# Autodesk Inventor assembly: Bio Assembly Skiba
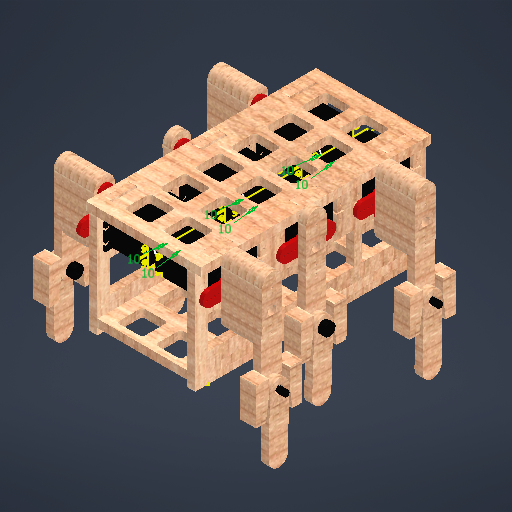
[picture p0: Inventor's stored thumbnail of the model, 512x512]
Saved by Autodesk Inventor 2026.2 (Build 302298000, 298)
## iProperties
Created: 2025-11-09
Part Number: Bio Assembly Skiba
Document SubType Name: Assembly
Designer: Nick
Author: Nick
## Documents named in this file (11)
- C:\Users\Nick\Downloads\CAD\Inventor\MMAE 232 Homeworks\Bio\Bio Assembly Skiba.iam
- C:\Users\Nick\Downloads\CAD\Inventor\MMAE 232 Homeworks\Bio\CAD Parts\Base-Skiba.ipt
- C:\Users\Nick\Downloads\CAD\Inventor\MMAE 232 Homeworks\Bio\CAD Parts\Servo Wall Skiba.ipt
- C:\Users\Nick\Downloads\CAD\Inventor\MMAE 232 Homeworks\Bio\CAD Parts\Bio Servo Skiba.ipt
- C:\Users\Nick\Downloads\CAD\Inventor\MMAE 232 Homeworks\Bio\CAD Parts\Servo Horn Skiba.ipt
- C:\Users\Nick\Downloads\CAD\Inventor\MMAE 232 Homeworks\Bio\CAD Parts\Roof Skiba.ipt
- C:\Users\Nick\Downloads\CAD\Inventor\MMAE 232 Homeworks\Bio\CAD Parts\Spacer Skiba.ipt
- C:\Users\Nick\Downloads\CAD\Inventor\MMAE 232 Homeworks\Bio\CAD Parts\Upper Leg Skiba.ipt
- C:\Users\Nick\Downloads\CAD\Inventor\MMAE 232 Homeworks\Bio\CAD Parts\Stop Skiba.ipt
- C:\Users\Nick\Downloads\CAD\Inventor\MMAE 232 Homeworks\Bio\CAD Parts\Lower Leg Skiba.ipt
- C:\Users\Nick\Downloads\CAD\Inventor\MMAE 232 Homeworks\Bio\CAD Parts\93897A255_Nylon Shoulder Screws (Short Screw) Skiba.ipt
## Components (62 placed, 10 different names)
1. Base-Skiba:1 — Flush:14, Mate:65, Flush:23, Flush:24, Flush:25, Flush:26, Mate:66
2. Servo Wall Skiba:1 — Mate:3, Mate:4, Mate:5, Mate:65, Flush:23, Flush:24, Flush:27, Mate:67, Flush:28
3. Servo Horn Skiba:2 — Mate:16, Mate:17, Mate:84, Mate:85, Mate:86
4. Servo Wall Skiba:2 — Flush:14, Mate:36, Mate:37, Mate:38, Flush:25, Flush:26, Mate:66
5. Servo Horn Skiba:5 — Mate:41, Mate:42, Mate:108, Mate:109, Mate:110
6. Roof Skiba:1 — Flush:27, Mate:67, Flush:28
7. Upper Leg Skiba:2 — Mate:84, Mate:85, Mate:86, Mate:87, Flush:35, Flush:36, Mate:88, Mate:89, Mate:117, Flush:47, Flush:48
8. Stop Skiba:2 — Mate:87, Flush:35, Flush:36
9. 93897A255_Nylon Shoulder Screws (Short Screw) Skiba:2 — Mate:90, Mate:91
10. Lower Leg Skiba:2 — Mate:88, Mate:89, Mate:90, Mate:91
11. Upper Leg Skiba:5 — Mate:108, Mate:109, Mate:110, Mate:111, Flush:43, Flush:44, Mate:112, Mate:113, Mate:120, Flush:53, Flush:54
12. Stop Skiba:5 — Mate:111, Flush:43, Flush:44
13. Lower Leg Skiba:5 — Mate:112, Mate:113, Mate:114, Mate:115
14. 93897A255_Nylon Shoulder Screws (Short Screw) Skiba:5 — Mate:114, Mate:115
15. Stop Skiba:7 — Mate:116, Flush:45, Flush:46
16. Stop Skiba:8 — Mate:117, Flush:47, Flush:48
17. Stop Skiba:9 — Mate:118, Flush:49, Flush:50
18. Stop Skiba:10 — Mate:119, Flush:51, Flush:52
19. Stop Skiba:11 — Mate:120, Flush:53, Flush:54
20. Stop Skiba:12 — Mate:121, Flush:55, Flush:56
21. Bio Servo Skiba:1 — Mate:3, Mate:4, Mate:5, Mate:6, Mate:7
22. Bio Servo Skiba:2 — Mate:16, Mate:17
23. Bio Servo Skiba:3
24. Bio Servo Skiba:4 — Mate:36, Mate:37, Mate:38, Mate:39, Mate:40
25. Bio Servo Skiba:5 — Mate:41, Mate:42
26. Bio Servo Skiba:6
27. Servo Horn Skiba:1 — Mate:6, Mate:7, Mate:74, Mate:75, Mate:76
28. Spacer Skiba:2 — Mate:68, Flush:29, Mate:69, Mate:70, Flush:30
29. Spacer Skiba:1 — Mate:68, Flush:29, Mate:69, Mate:71, Mate:73, Mate:75
30. Upper Leg Skiba:1 — Mate:77, Mate:78, Flush:32, Mate:79, Flush:33, Flush:34, Mate:80, Mate:81, Mate:82, Mate:116, Flush:45, Flush:46
31. Spacer Skiba:4 — Mate:72, Flush:31, Mate:73, Mate:74, Mate:76, Mate:77, Mate:78, Flush:32
32. Spacer Skiba:3 — Mate:70, Flush:30, Mate:71, Mate:72, Flush:31
33. 93897A255_Nylon Shoulder Screws (Short Screw) Skiba:1 — Mate:82, Mate:83
34. Lower Leg Skiba:1 — Mate:80, Mate:81, Mate:83
35. Stop Skiba:1 — Mate:79, Flush:33, Flush:34
36. Servo Horn Skiba:6
37. Spacer Skiba:5
38. Spacer Skiba:6
39. Upper Leg Skiba:3 — Mate:118, Flush:49, Flush:50
40. Spacer Skiba:7
41. Spacer Skiba:8
42. 93897A255_Nylon Shoulder Screws (Short Screw) Skiba:3
43. Lower Leg Skiba:3
44. Stop Skiba:3
45. Spacer Skiba:9 — Mate:92, Mate:93, Mate:94, Mate:95, Mate:96, Flush:37
46. Spacer Skiba:11 — Mate:95, Mate:96, Flush:37, Mate:97, Mate:98, Flush:38
47. Spacer Skiba:10 — Mate:97, Mate:98, Flush:38, Mate:99, Mate:100, Flush:39
48. Spacer Skiba:12 — Mate:99, Mate:100, Flush:39, Mate:101, Mate:102, Flush:40
49. Upper Leg Skiba:4 — Mate:101, Mate:102, Flush:40, Mate:103, Flush:41, Flush:42, Mate:104, Mate:105, Mate:106, Mate:119, Flush:51, Flush:52
50. 93897A255_Nylon Shoulder Screws (Short Screw) Skiba:4 — Mate:106, Mate:107
51. Stop Skiba:4 — Mate:103, Flush:41, Flush:42
52. Lower Leg Skiba:4 — Mate:104, Mate:105, Mate:107
53. Servo Horn Skiba:4 — Mate:39, Mate:40, Mate:92, Mate:93, Mate:94
54. Spacer Skiba:13
55. Spacer Skiba:14
56. Spacer Skiba:15
57. Spacer Skiba:16
58. Upper Leg Skiba:6 — Mate:121, Flush:55, Flush:56
59. 93897A255_Nylon Shoulder Screws (Short Screw) Skiba:6
60. Stop Skiba:6
61. Lower Leg Skiba:6
62. Servo Horn Skiba:7
## Component patterns: (3 elements, first: Bio Servo Skiba:1), (3 elements, first: Bio Servo Skiba:4), (2 elements, first: Servo Horn Skiba:1 + Spacer Skiba:2 + Spacer Skiba:1 + Upper Leg Skiba:1 + Spacer Skiba:4 + Spacer Skiba:3 + 93897A255_Nylon Shoulder Screws (Short Screw) Skiba:1 + Lower Leg Skiba:1 + Stop Skiba:1), (2 elements, first: Spacer Skiba:9 + Spacer Skiba:11 + Spacer Skiba:10 + Spacer Skiba:12 + Upper Leg Skiba:4 + 93897A255_Nylon Shoulder Screws (Short Screw) Skiba:4 + Stop Skiba:4 + Lower Leg Skiba:4 + Servo Horn Skiba:4)
## Relationships (106: Mate 71, Flush 35)
- Mate:3: Servo Wall Skiba:1 ↔ Bio Servo Skiba:1
- Mate:4: Servo Wall Skiba:1 ↔ Bio Servo Skiba:1
- Mate:5: Servo Wall Skiba:1 ↔ Bio Servo Skiba:1
- Mate:6: Bio Servo Skiba:1 ↔ Servo Horn Skiba:1
- Mate:7: Bio Servo Skiba:1 ↔ Servo Horn Skiba:1
- Mate:16: Servo Horn Skiba:2 ↔ Bio Servo Skiba:2
- Mate:17: Servo Horn Skiba:2 ↔ Bio Servo Skiba:2
- Flush:14: Base-Skiba:1 ↔ Servo Wall Skiba:2
- Mate:36: Servo Wall Skiba:2 ↔ Bio Servo Skiba:4
- Mate:37: Servo Wall Skiba:2 ↔ Bio Servo Skiba:4
- Mate:38: Servo Wall Skiba:2 ↔ Bio Servo Skiba:4
- Mate:39: Bio Servo Skiba:4 ↔ Servo Horn Skiba:4
- Mate:40: Bio Servo Skiba:4 ↔ Servo Horn Skiba:4
- Mate:41: Servo Horn Skiba:5 ↔ Bio Servo Skiba:5
- Mate:42: Servo Horn Skiba:5 ↔ Bio Servo Skiba:5
- Mate:65: Base-Skiba:1 ↔ Servo Wall Skiba:1
- Flush:23: Base-Skiba:1 ↔ Servo Wall Skiba:1
- Flush:24: Base-Skiba:1 ↔ Servo Wall Skiba:1
- Flush:25: Base-Skiba:1 ↔ Servo Wall Skiba:2
- Flush:26: Base-Skiba:1 ↔ Servo Wall Skiba:2
- Mate:66: Base-Skiba:1 ↔ Servo Wall Skiba:2
- Flush:27: Servo Wall Skiba:1 ↔ Roof Skiba:1
- Mate:67: Servo Wall Skiba:1 ↔ Roof Skiba:1
- Flush:28: Servo Wall Skiba:1 ↔ Roof Skiba:1
- Mate:68: Spacer Skiba:2 ↔ Spacer Skiba:1
- Flush:29: Spacer Skiba:2 ↔ Spacer Skiba:1
- Mate:69: Spacer Skiba:2 ↔ Spacer Skiba:1
- Mate:70: Spacer Skiba:2 ↔ Spacer Skiba:3
- Flush:30: Spacer Skiba:2 ↔ Spacer Skiba:3
- Mate:71: Spacer Skiba:1 ↔ Spacer Skiba:3
- Mate:72: Spacer Skiba:4 ↔ Spacer Skiba:3
- Flush:31: Spacer Skiba:4 ↔ Spacer Skiba:3
- Mate:73: Spacer Skiba:1 ↔ Spacer Skiba:4
- Mate:74: Servo Horn Skiba:1 ↔ Spacer Skiba:4
- Mate:75: Servo Horn Skiba:1 ↔ Spacer Skiba:1
- Mate:76: Servo Horn Skiba:1 ↔ Spacer Skiba:4
- Mate:77: Upper Leg Skiba:1 ↔ Spacer Skiba:4
- Mate:78: Upper Leg Skiba:1 ↔ Spacer Skiba:4
- Flush:32: Upper Leg Skiba:1 ↔ Spacer Skiba:4
- Mate:79: Upper Leg Skiba:1 ↔ Stop Skiba:1
- Flush:33: Upper Leg Skiba:1 ↔ Stop Skiba:1
- Flush:34: Upper Leg Skiba:1 ↔ Stop Skiba:1
- Mate:80: Upper Leg Skiba:1 ↔ Lower Leg Skiba:1
- Mate:81: Upper Leg Skiba:1 ↔ Lower Leg Skiba:1
- Mate:82: Upper Leg Skiba:1 ↔ 93897A255_Nylon Shoulder Screws (Short Screw) Skiba:1
- Mate:83: 93897A255_Nylon Shoulder Screws (Short Screw) Skiba:1 ↔ Lower Leg Skiba:1
- Mate:84: Servo Horn Skiba:2 ↔ Upper Leg Skiba:2
- Mate:85: Servo Horn Skiba:2 ↔ Upper Leg Skiba:2
- Mate:86: Servo Horn Skiba:2 ↔ Upper Leg Skiba:2
- Mate:87: Upper Leg Skiba:2 ↔ Stop Skiba:2
- Flush:35: Upper Leg Skiba:2 ↔ Stop Skiba:2
- Flush:36: Upper Leg Skiba:2 ↔ Stop Skiba:2
- Mate:88: Upper Leg Skiba:2 ↔ Lower Leg Skiba:2
- Mate:89: Upper Leg Skiba:2 ↔ Lower Leg Skiba:2
- Mate:90: 93897A255_Nylon Shoulder Screws (Short Screw) Skiba:2 ↔ Lower Leg Skiba:2
- Mate:91: 93897A255_Nylon Shoulder Screws (Short Screw) Skiba:2 ↔ Lower Leg Skiba:2
- Mate:92: Spacer Skiba:9 ↔ Servo Horn Skiba:4
- Mate:93: Spacer Skiba:9 ↔ Servo Horn Skiba:4
- Mate:94: Spacer Skiba:9 ↔ Servo Horn Skiba:4
- Mate:95: Spacer Skiba:9 ↔ Spacer Skiba:11
- Mate:96: Spacer Skiba:9 ↔ Spacer Skiba:11
- Flush:37: Spacer Skiba:9 ↔ Spacer Skiba:11
- Mate:97: Spacer Skiba:11 ↔ Spacer Skiba:10
- Mate:98: Spacer Skiba:11 ↔ Spacer Skiba:10
- Flush:38: Spacer Skiba:11 ↔ Spacer Skiba:10
- Mate:99: Spacer Skiba:10 ↔ Spacer Skiba:12
- Mate:100: Spacer Skiba:10 ↔ Spacer Skiba:12
- Flush:39: Spacer Skiba:10 ↔ Spacer Skiba:12
- Mate:101: Spacer Skiba:12 ↔ Upper Leg Skiba:4
- Mate:102: Spacer Skiba:12 ↔ Upper Leg Skiba:4
- Flush:40: Spacer Skiba:12 ↔ Upper Leg Skiba:4
- Mate:103: Upper Leg Skiba:4 ↔ Stop Skiba:4
- Flush:41: Upper Leg Skiba:4 ↔ Stop Skiba:4
- Flush:42: Upper Leg Skiba:4 ↔ Stop Skiba:4
- Mate:104: Upper Leg Skiba:4 ↔ Lower Leg Skiba:4
- Mate:105: Upper Leg Skiba:4 ↔ Lower Leg Skiba:4
- Mate:106: Upper Leg Skiba:4 ↔ 93897A255_Nylon Shoulder Screws (Short Screw) Skiba:4
- Mate:107: 93897A255_Nylon Shoulder Screws (Short Screw) Skiba:4 ↔ Lower Leg Skiba:4
- Mate:108: Servo Horn Skiba:5 ↔ Upper Leg Skiba:5
- Mate:109: Servo Horn Skiba:5 ↔ Upper Leg Skiba:5
- Mate:110: Servo Horn Skiba:5 ↔ Upper Leg Skiba:5
- Mate:111: Upper Leg Skiba:5 ↔ Stop Skiba:5
- Flush:43: Upper Leg Skiba:5 ↔ Stop Skiba:5
- Flush:44: Upper Leg Skiba:5 ↔ Stop Skiba:5
- Mate:112: Upper Leg Skiba:5 ↔ Lower Leg Skiba:5
- Mate:113: Upper Leg Skiba:5 ↔ Lower Leg Skiba:5
- Mate:114: Lower Leg Skiba:5 ↔ 93897A255_Nylon Shoulder Screws (Short Screw) Skiba:5
- Mate:115: Lower Leg Skiba:5 ↔ 93897A255_Nylon Shoulder Screws (Short Screw) Skiba:5
- Mate:116: Stop Skiba:7 ↔ Upper Leg Skiba:1
- Flush:45: Stop Skiba:7 ↔ Upper Leg Skiba:1
- Flush:46: Stop Skiba:7 ↔ Upper Leg Skiba:1
- Mate:117: Upper Leg Skiba:2 ↔ Stop Skiba:8
- Flush:47: Upper Leg Skiba:2 ↔ Stop Skiba:8
- Flush:48: Upper Leg Skiba:2 ↔ Stop Skiba:8
- Mate:118: Stop Skiba:9 ↔ Upper Leg Skiba:3
- Flush:49: Stop Skiba:9 ↔ Upper Leg Skiba:3
- Flush:50: Stop Skiba:9 ↔ Upper Leg Skiba:3
- Mate:119: Stop Skiba:10 ↔ Upper Leg Skiba:4
- Flush:51: Stop Skiba:10 ↔ Upper Leg Skiba:4
- Flush:52: Stop Skiba:10 ↔ Upper Leg Skiba:4
- Mate:120: Upper Leg Skiba:5 ↔ Stop Skiba:11
- Flush:53: Upper Leg Skiba:5 ↔ Stop Skiba:11
- Flush:54: Upper Leg Skiba:5 ↔ Stop Skiba:11
- Mate:121: Stop Skiba:12 ↔ Upper Leg Skiba:6
- Flush:55: Stop Skiba:12 ↔ Upper Leg Skiba:6
- Flush:56: Stop Skiba:12 ↔ Upper Leg Skiba:6
